# Autodesk Inventor assembly: Display
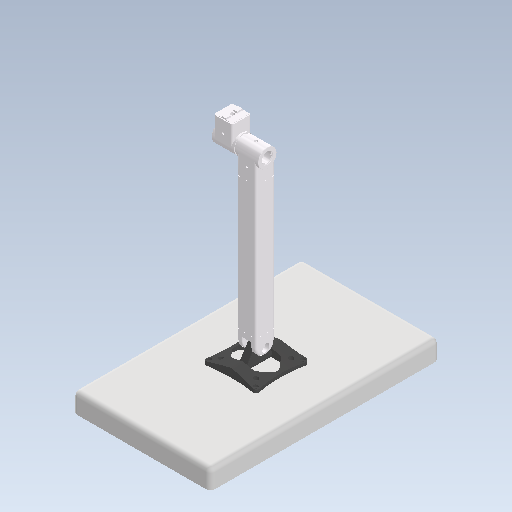
[picture p0: Inventor's stored thumbnail of the model, 512x512]
Saved by Autodesk Inventor 2020 (Build 240168000, 168)
## iProperties
Created: 2019-11-09
Part Number: Display
Document SubType Name: Assembly
Designer: nicoc
Author: nicoc
## Documents named in this file (3)
- D:\03_Bachelor\Semester_5\pro5E\Stand\CAD\Version2\Display\Display.iam
- D:\03_Bachelor\Semester_5\pro5E\Stand\CAD\Version2\Display\MonitorHolder\item_0064944_Monitor_Arm_A1=0_A2=0_A3=0_1.iam
- D:\03_Bachelor\Semester_5\pro5E\Stand\CAD\Version2\Display\Monitor.ipt
## Components (2 placed, 2 different names)
1. item_0064944_Monitor_Arm_A1=0_A2=0_A3=0_1:1 [sub-assembly] — Mate:1, Mate:2, Mate:3
2. Monitor:1 — Mate:1, Mate:2, Mate:3
## Relationships (3: Mate 3)
- Mate:1: item_0064944_Monitor_Arm_A1=0_A2=0_A3=0_1:1 ↔ Monitor:1
- Mate:2: item_0064944_Monitor_Arm_A1=0_A2=0_A3=0_1:1 ↔ Monitor:1
- Mate:3: item_0064944_Monitor_Arm_A1=0_A2=0_A3=0_1:1 ↔ Monitor:1
